# Autodesk Inventor assembly: AN929-8D
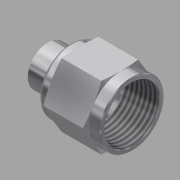
[picture p0: Inventor's stored thumbnail of the model, 180x180]
Saved by Autodesk Inventor 2019 (Build 230136000, 136)
## iProperties
Created: 2018-11-23
Part Number: AN929-8D
Document SubType Name: Assembly
Designer: erics
Mass: 17.068 g
Surface Area: 47.3629 cm^2
Volume: 6.11916 cm^3
Density: 2.78927 g/cm^3
Author: erics
## Documents named in this file (18)
- D:\Users\erics\Documents\CAD Library\Pipe Fittings\AN-MS-Fittings\AN929.iam
- D:\Users\erics\Documents\CAD Library\Pipe Fittings\AN-MS-Fittings\AN929\AN929-8D.ipt
- D:\Users\erics\Documents\CAD Library\Pipe Fittings\AN-MS-Fittings\AN929.ipt
- D:\Users\erics\Documents\CAD Library\Pipe Fittings\AN-MS-Fittings\AN818.ipt
- D:\Users\erics\Documents\CAD Library\Pipe Fittings\AN-MS-Fittings\AN818\AN818-8D.ipt
- AN929-10D.iam
- AN929-12D.iam
- AN929-16D.iam
- AN929-20D.iam
- AN929-24D.iam
- AN929-28D.iam
- AN929-2D.iam
- AN929-32D.iam
- AN929-3D.iam
- AN929-4D.iam
- AN929-5D.iam
- AN929-6D.iam
- AN929-8D.iam
## Components (2 placed, 2 different names)
1. AN929-8D:1 — Insert:1
2. AN818-8D:1 — Insert:1
## Relationships (1: Insert 1)
- Insert:1: AN929-8D:1 ↔ AN818-8D:1
